# Autodesk Inventor assembly: HS-755MG_ASM
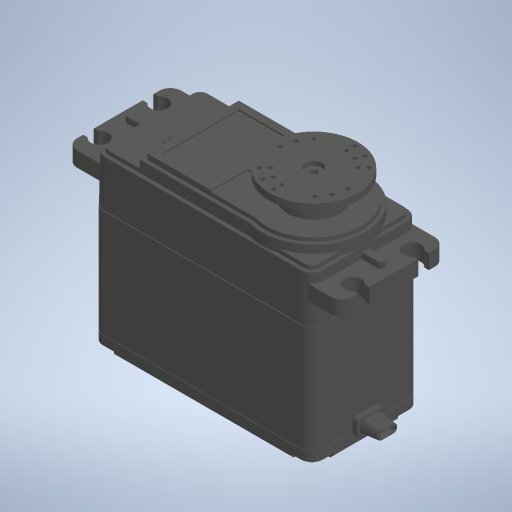
[picture p0: Inventor's stored thumbnail of the model, 512x512]
Saved by Autodesk Inventor 2024 (Build 280153000, 153)
## iProperties
Created: 2017-08-30
Part Number: HS-755MG_ASM
Document SubType Name: Assembly
Designer: johnn
Sending System: CREO PARAMETRIC BY PTC INC, 2014440
Preprocessor: CREO PARAMETRIC BY PTC INC, 2014440
Title: HS-755MG_ASM
Author: servo-csw
Revision Number: 1LAST_VERSION
## Documents named in this file (3)
- E:\TRACER DOCUMENTS\SheetMetal\Servo 775 (with Spline).iam
- E:\TRACER DOCUMENTS\SheetMetal\HS-755MG-1643916399\_HS-755MG.ipt
- E:\TRACER DOCUMENTS\SheetMetal\Round Micro Servo Horn.ipt
## Components (2 placed, 2 different names)
1. 51 — Mate:1, Mate:2
2. Round Micro Servo Horn:1 — Mate:1, Mate:2
## Relationships (2: Mate 2)
- Mate:1: 51 ↔ Round Micro Servo Horn:1
- Mate:2: 51 ↔ Round Micro Servo Horn:1
